# Autodesk Inventor assembly: Speaker Clamp Assembly
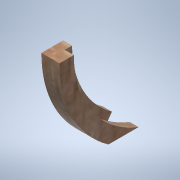
[picture p0: Inventor's stored thumbnail of the model, 180x180]
Saved by Autodesk Inventor 2021 (Build 250183000, 183)
## iProperties
Created: 2017-12-06
Part Number: Speaker Clamp Assembly
Document SubType Name: Assembly
Designer: Andrew
Author: Andrew
## Documents named in this file (3)
- D:\OneDrive\3D Models\AM Radio\Speaker Clamp Assembly.iam
- D:\OneDrive\3D Models\AM Radio\Speaker Clamp Back.ipt
- D:\OneDrive\3D Models\AM Radio\Speaker Clamp.ipt
## Components (2 placed, 2 different names)
1. Speaker Clamp Back:1 — Mate:1, Mate:2, Flush:1
2. Speaker Clamp:1 — Mate:1, Mate:2, Flush:1
## Relationships (3: Mate 2, Flush 1)
- Mate:1: Speaker Clamp Back:1 ↔ Speaker Clamp:1
- Mate:2: Speaker Clamp Back:1 ↔ Speaker Clamp:1
- Flush:1: Speaker Clamp Back:1 ↔ Speaker Clamp:1
